# Autodesk Inventor assembly: end room with super computer
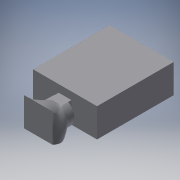
[picture p0: Inventor's stored thumbnail of the model, 180x180]
Saved by Autodesk Inventor 2017 (Build 210142000, 142)
## iProperties
Created: 2018-04-23
Part Number: end room with super computer
Document SubType Name: Assembly
Designer: braxtonwright
Author: braxtonwright
## Documents named in this file (4)
- E:\School\Game develpment\geoscape\done\single wall\map (one wall)\end room with super computer.iam
- E:\School\Game develpment\geoscape\done\single wall\rooms  (one wall)\end room.ipt
- E:\School\Game develpment\geoscape\done\single wall\rooms  (one wall)\end room super computer.ipt
- E:\School\Game develpment\geoscape\done\single wall\doors (one wall)\9 foot door (one wall)\(closed face) end door room (one wall) (9).ipt
## Components (3 placed, 3 different names)
1. end room:1 — Mate:1, Mate:2, Mate:3, Insert:1, Flush:1
2. end room super computer:1 — Mate:1, Mate:2, Mate:3
3. (closed face) end door room (one wall) (9):1 — Insert:1, Flush:1
## Relationships (5: Mate 3, Insert 1, Flush 1)
- Mate:1: end room:1 ↔ end room super computer:1
- Mate:2: end room:1 ↔ end room super computer:1
- Mate:3: end room:1 ↔ end room super computer:1
- Insert:1: end room:1 ↔ (closed face) end door room (one wall) (9):1
- Flush:1: end room:1 ↔ (closed face) end door room (one wall) (9):1
